# Autodesk Inventor assembly: Drivebox_MIR
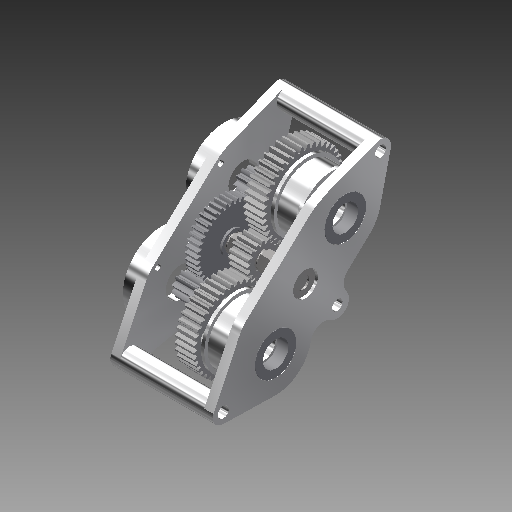
[picture p0: Inventor's stored thumbnail of the model, 512x512]
Saved by Autodesk Inventor 2019.4 (Build 234330000, 330)
## iProperties
Created: 2020-01-05
Part Number: Drivebox_MIR
Document SubType Name: Assembly
Designer: Mark
Mass: 1259.19 g
Surface Area: 1354.77 cm^2
Volume: 329.889 cm^3
Density: 3.81702 g/cm^3
Author: Mark
## Documents named in this file (13)
- C:\Users\Mark\Desktop\7738 Helion Engineering\7738-2020\CAD\Gearbox\Drivebox_MIR.iam
- C:\Users\Mark\Desktop\7738 Helion Engineering\7738-2020\CAD\Gearbox\Gearbox Plate 1_MIR.ipt
- C:\Users\Mark\Desktop\7738 Helion Engineering\7738-2020\CAD\Gearbox\Gearbox Plate 2_MIR.ipt
- C:\Users\Mark\Desktop\7738 Helion Engineering\7738-2020\CAD\Gearbox\Shaft Jr_MIR.ipt
- C:\Users\Mark\Desktop\7738 Helion Engineering\7738-2020\CAD\Gearbox\F6800_MIR.ipt
- C:\Users\Mark\Desktop\7738 Helion Engineering\7738-2020\CAD\Gearbox\Spacer_MIR.ipt
- C:\Users\Mark\Desktop\7738 Helion Engineering\7738-2020\CAD\Gearbox\F6804_MIR.ipt
- C:\Users\Mark\Desktop\7738 Helion Engineering\7738-2020\CAD\Gearbox\10T_Steel_Spur_Gear_20_DP_12T_Center_Distance_Falcon_Motor_217-6917_MIR.ipt
- C:\Users\Mark\Desktop\7738 Helion Engineering\7738-2020\CAD\Gearbox\40t_Aluminum_Spur_Gear_20_DP_1_2_Hex_Bore_217-2708_MIR.ipt
- C:\Users\Mark\Desktop\7738 Helion Engineering\7738-2020\CAD\Gearbox\Gearbox\Design Accelerator\Spur Gears1_MIR1.iam
- C:\Users\Mark\Desktop\7738 Helion Engineering\7738-2020\CAD\Gearbox\Gearbox\Design Accelerator\Spur Gears2_MIR1.iam
- C:\Users\Mark\Desktop\7738 Helion Engineering\7738-2020\CAD\Gearbox\HTD 5M 30 20mm ID Keyed_MIR.ipt
- C:\Users\Mark\Desktop\7738 Helion Engineering\7738-2020\CAD\Motor Spacer_MIR.ipt
## Components (19 placed, 12 different names)
1. Gearbox Plate 1_MIR:1 — Flush:3, Mate:4, Mate:3, Mate:45, Mate:47, Mate:46, Mate:14, Mate:13, Mate:25, Mate:26, Mate:43, Mate:54, Mate:56
2. Gearbox Plate 2_MIR:1 — Flush:3, Mate:39, Mate:38, Mate:37, Mate:44, Mate:34, Mate:33, Mate:36, Mate:35, Mate:40, Mate:49, Mate:51
3. Shaft Jr_MIR:1 — Mate:8, Mate:7, Mate:41
4. F6800_MIR:1 — Mate:39, Mate:8, Mate:7, Mate:4, Mate:3, Mate:42
5. F6800_MIR:2 — Mate:41, Mate:38, Mate:37
6. Spacer_MIR:1 — Mate:44, Mate:45
7. Spacer_MIR:2 — Mate:47, Mate:46
8. Spacer_MIR:3 — Mate:14, Mate:13
9. F6804_MIR:1 — Mate:34, Mate:33, Mate:31, Mate:50
10. F6804_MIR:2 — Mate:36, Mate:35, Mate:32, Mate:48
11. 10T_Steel_Spur_Gear_20_DP_12T_Center_Distance_Falcon_Motor_217-6917_MIR:1 — Mate:25
12. 10T_Steel_Spur_Gear_20_DP_12T_Center_Distance_Falcon_Motor_217-6917_MIR:2 — Mate:26
13. 40t_Aluminum_Spur_Gear_20_DP_1_2_Hex_Bore_217-2708_MIR:1 — Mate:43, Mate:42, Mate:30
14. Spur Gears1_MIR1:1 [sub-assembly] — Mate:40, Mate:31, Mate:30, Flush:2
15. Spur Gears2_MIR1:1 [sub-assembly] — Flush:2, Mate:32
16. HTD 5M 30 20mm ID Keyed_MIR:1 — Mate:49, Mate:48
17. HTD 5M 30 20mm ID Keyed_MIR:2 — Mate:51, Mate:50
18. Motor Spacer_MIR:1 — Mate:54
19. Motor Spacer_MIR:2 — Mate:56
## Relationships (34: Mate 32, Flush 2)
- Flush:3: Gearbox Plate 1_MIR:1 ↔ Gearbox Plate 2_MIR:1
- Mate:39: Gearbox Plate 2_MIR:1 ↔ F6800_MIR:1
- Mate:8 (0.2 mm): Shaft Jr_MIR:1 ↔ F6800_MIR:1
- Mate:7: Shaft Jr_MIR:1 ↔ F6800_MIR:1
- Mate:4: Gearbox Plate 1_MIR:1 ↔ F6800_MIR:1
- Mate:3: Gearbox Plate 1_MIR:1 ↔ F6800_MIR:1
- Mate:41 (0.2 mm): Shaft Jr_MIR:1 ↔ F6800_MIR:2
- Mate:38: Gearbox Plate 2_MIR:1 ↔ F6800_MIR:2
- Mate:37: Gearbox Plate 2_MIR:1 ↔ F6800_MIR:2
- Mate:44: Gearbox Plate 2_MIR:1 ↔ Spacer_MIR:1
- Mate:45: Gearbox Plate 1_MIR:1 ↔ Spacer_MIR:1
- Mate:47: Gearbox Plate 1_MIR:1 ↔ Spacer_MIR:2
- Mate:46: Gearbox Plate 1_MIR:1 ↔ Spacer_MIR:2
- Mate:14: Gearbox Plate 1_MIR:1 ↔ Spacer_MIR:3
- Mate:13: Gearbox Plate 1_MIR:1 ↔ Spacer_MIR:3
- Mate:34: Gearbox Plate 2_MIR:1 ↔ F6804_MIR:1
- Mate:33: Gearbox Plate 2_MIR:1 ↔ F6804_MIR:1
- Mate:36: Gearbox Plate 2_MIR:1 ↔ F6804_MIR:2
- Mate:35: Gearbox Plate 2_MIR:1 ↔ F6804_MIR:2
- Mate:25 (1 mm): Gearbox Plate 1_MIR:1 ↔ 10T_Steel_Spur_Gear_20_DP_12T_Center_Distance_Falcon_Motor_217-6917_MIR:1
- Mate:26 (1 mm): Gearbox Plate 1_MIR:1 ↔ 10T_Steel_Spur_Gear_20_DP_12T_Center_Distance_Falcon_Motor_217-6917_MIR:2
- Mate:43 (4 mm): Gearbox Plate 1_MIR:1 ↔ 40t_Aluminum_Spur_Gear_20_DP_1_2_Hex_Bore_217-2708_MIR:1
- Mate:42: F6800_MIR:1 ↔ 40t_Aluminum_Spur_Gear_20_DP_1_2_Hex_Bore_217-2708_MIR:1
- Mate:40: Gearbox Plate 2_MIR:1 ↔ Spur Gears1_MIR1:1
- Mate:31: F6804_MIR:1 ↔ Spur Gears1_MIR1:1
- Mate:30 (8 mm): 40t_Aluminum_Spur_Gear_20_DP_1_2_Hex_Bore_217-2708_MIR:1 ↔ Spur Gears1_MIR1:1
- Flush:2: Spur Gears1_MIR1:1 ↔ Spur Gears2_MIR1:1
- Mate:32: F6804_MIR:2 ↔ Spur Gears2_MIR1:1
- Mate:49 (3 mm): Gearbox Plate 2_MIR:1 ↔ HTD 5M 30 20mm ID Keyed_MIR:1
- Mate:48: F6804_MIR:2 ↔ HTD 5M 30 20mm ID Keyed_MIR:1
- Mate:51 (3 mm): Gearbox Plate 2_MIR:1 ↔ HTD 5M 30 20mm ID Keyed_MIR:2
- Mate:50: F6804_MIR:1 ↔ HTD 5M 30 20mm ID Keyed_MIR:2
- Mate:54: Gearbox Plate 1_MIR:1 ↔ Motor Spacer_MIR:1
- Mate:56: Gearbox Plate 1_MIR:1 ↔ Motor Spacer_MIR:2
